# Autodesk Inventor assembly: end room with super computer
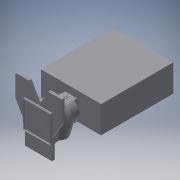
[picture p0: Inventor's stored thumbnail of the model, 180x180]
Saved by Autodesk Inventor 2017 (Build 210142000, 142)
## iProperties
Created: 2018-04-23
Part Number: end room with super computer
Document SubType Name: Assembly
Designer: braxtonwright
Author: braxtonwright
## Documents named in this file (6)
- E:\School\Game develpment\geoscape\rooms\assemblys\end room with super computer.iam
- E:\School\Game develpment\geoscape\rooms\end room.ipt
- E:\School\Game develpment\geoscape\rooms\end room super computer.ipt
- E:\School\Game develpment\geoscape\done (one wall)\doors\end door (one wall)\9 foot door\end door room (9).ipt
- E:\School\Game develpment\geoscape\done (one wall)\doors\end door (one wall)\9 foot door\end door assembly (closed) (9).ipt.iam
- end door assembly (closed) (9).ipt
## Components (4 placed, 4 different names)
1. end room:1 — Mate:1, Mate:2, Mate:3, Flush:1, Insert:1
2. end room super computer:1 — Mate:1, Mate:2, Mate:3
3. end door room (9):1 — Flush:1, Insert:1, Mate:4, Mate:5
4. end door assembly (closed) (9).ipt:1 [sub-assembly] — Mate:4, Mate:5
## Relationships (7: Mate 5, Flush 1, Insert 1)
- Mate:1: end room:1 ↔ end room super computer:1
- Mate:2: end room:1 ↔ end room super computer:1
- Mate:3: end room:1 ↔ end room super computer:1
- Flush:1: end room:1 ↔ end door room (9):1
- Insert:1: end room:1 ↔ end door room (9):1
- Mate:4: end door room (9):1 ↔ end door assembly (closed) (9).ipt:1
- Mate:5: end door room (9):1 ↔ end door assembly (closed) (9).ipt:1
